# Autodesk Inventor assembly: 210mmPost
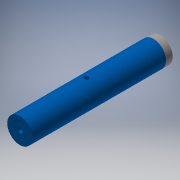
[picture p0: Inventor's stored thumbnail of the model, 180x180]
Saved by Autodesk Inventor 2016 (Build 200138000, 138)
## iProperties
Created: 2016-04-07
Part Number: 210mmPost
Document SubType Name: Assembly
Designer: sims01
Author: sims01
## Documents named in this file (3)
- H:\Documents\LSFM_3\setup\mechanical\design\lsfm3_mechDesignMar16\210mmPost.iam
- H:\Documents\LSFM_3\setup\mechanical\design\lsfm3_mechDesignMar16\200mmPost.ipt
- H:\Documents\LSFM_3\setup\mechanical\design\lsfm3_mechDesignMar16\10mmPostSpacer.ipt
## Components (2 placed, 2 different names)
1. 200mmPost:1 — Rigid:1
2. 10mmPostSpacer:1 — Rigid:1
## Relationships (1: WeldJoint 1)
- Rigid:1 [WeldJoint]: 200mmPost:1 ↔ 10mmPostSpacer:1
